# Autodesk Inventor assembly: Nozzle 8-inch v1
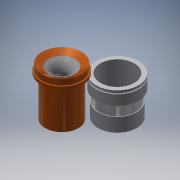
[picture p0: Inventor's stored thumbnail of the model, 180x180]
Saved by Autodesk Inventor 2017 (Build 210142000, 142)
## iProperties
Created: 2016-07-10
Part Number: Nozzle 8-inch v1
Document SubType Name: Assembly
Designer: Bill
Author: Bill
## Documents named in this file (6)
- C:\Users\Bill\Desktop\Propulsion\Launches\8-inch-flight\Design\CAD Files\trunk\Version 1\Nozzle 8-inch v1.iam
- C:\Users\Bill\Desktop\Propulsion\Launches\8-inch-flight\Design\CAD Files\trunk\Version 1\Aluminum Carrier 8-inch v1.ipt
- C:\Users\Bill\Desktop\Propulsion\Launches\8-inch-flight\Design\CAD Files\trunk\Version 1\Aluminum Retainer 8-inch v1.ipt
- C:\Users\Bill\Desktop\Propulsion\Launches\8-inch-flight\Design\CAD Files\trunk\Version 1\Aluminum Skirt 8-inch v1.ipt
- C:\Users\Bill\Desktop\Propulsion\Launches\8-inch-flight\Design\CAD Files\trunk\Version 1\Graphite 8-inch v1.ipt
- C:\Users\Bill\Desktop\Propulsion\Launches\8-inch-flight\Design\CAD Files\trunk\Version 1\Phenolic 8-inch v1.ipt
## Components (5 placed, 5 different names)
1. Aluminum Carrier 8-inch v1:1 — Mate:1, Mate:2, Mate:3, Mate:4
2. Aluminum Retainer 8-inch v1:1 — Mate:1, Mate:2
3. Aluminum Skirt 8-inch v1:1 — Mate:3, Mate:4
4. Graphite 8-inch v1:1 — Mate:5, Mate:6
5. Phenolic 8-inch v1:1 — Mate:5, Mate:6
## Relationships (6: Mate 6)
- Mate:1: Aluminum Carrier 8-inch v1:1 ↔ Aluminum Retainer 8-inch v1:1
- Mate:2: Aluminum Carrier 8-inch v1:1 ↔ Aluminum Retainer 8-inch v1:1
- Mate:3: Aluminum Carrier 8-inch v1:1 ↔ Aluminum Skirt 8-inch v1:1
- Mate:4: Aluminum Carrier 8-inch v1:1 ↔ Aluminum Skirt 8-inch v1:1
- Mate:5: Graphite 8-inch v1:1 ↔ Phenolic 8-inch v1:1
- Mate:6: Graphite 8-inch v1:1 ↔ Phenolic 8-inch v1:1
